# Autodesk Inventor assembly: Robot Assembly MK2
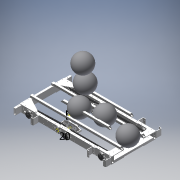
[picture p0: Inventor's stored thumbnail of the model, 180x180]
Saved by Autodesk Inventor 2019.4 (Build 234330000, 330)
## iProperties
Created: 2020-01-18
Part Number: Robot Assembly MK2
Document SubType Name: Assembly
Designer: Mark
Author: Mark
## Documents named in this file (3)
- C:\Users\Mark\Desktop\7738 Helion Engineering\7738-2020\Robot Assembly MK2.iam
- C:\Users\Mark\Desktop\7738 Helion Engineering\7738-2020\CAD\Drivebase.iam
- C:\Users\Mark\Desktop\7738 Helion Engineering\7738-2020\Upper Stage\Upper Stage.iam
## Components (2 placed, 2 different names)
1. Drivebase:1 [sub-assembly] — Mate:1, Flush:1, Flush:2
2. Upper Stage:1 [sub-assembly] — Mate:1, Flush:1, Flush:2
## Relationships (3: Flush 2, Mate 1)
- Mate:1: Drivebase:1 ↔ Upper Stage:1
- Flush:1: Drivebase:1 ↔ Upper Stage:1
- Flush:2: Drivebase:1 ↔ Upper Stage:1
